# Autodesk Inventor assembly: Braço_robô_001
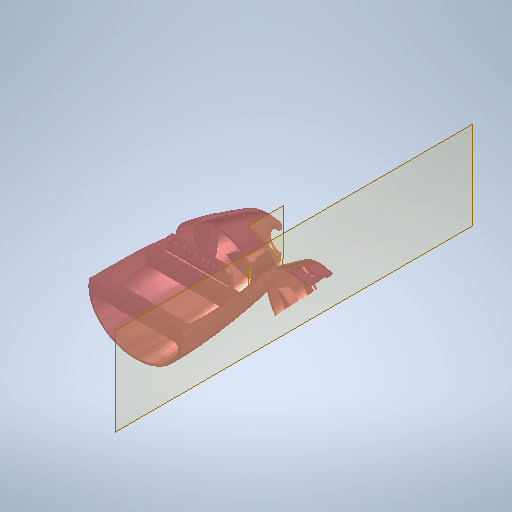
[picture p0: Inventor's stored thumbnail of the model, 512x512]
Saved by Autodesk Inventor 2025.2 (Build 292293000, 293)
## iProperties
Created: 2025-05-29
Part Number: Braço_robô_001
Document SubType Name: Assembly
Designer: Formação
Author: Formação
## Documents named in this file (8)
- C:\Users\Formação\Documents\Inventor\Mão_Robô_EMG\Mão Robótica 2.0\Braço_robô_001.iam
- C:\Users\Formação\Documents\Inventor\Mão_Robô_EMG\Mão Robótica 2.0\Braço\Mid Forearm Large.ipt
- C:\Users\Formação\Documents\Inventor\Mão_Robô_EMG\Mão Robótica 2.0\Braço\Mid Forearm Small.ipt
- C:\Users\Formação\Documents\Inventor\Mão_Robô_EMG\Mão Robótica 2.0\Braço\wrist clearance A.ipt
- C:\Users\Formação\Documents\Inventor\Mão_Robô_EMG\Mão Robótica 2.0\Braço\wrist clearance B.ipt
- C:\Users\Formação\Documents\Inventor\Mão_Robô_EMG\Mão Robótica 2.0\Braço\Wrist Forearm Section A.ipt
- C:\Users\Formação\Documents\Inventor\Mão_Robô_EMG\Mão Robótica 2.0\Braço\Wrist Forearm Section B.ipt
- C:\Users\Formação\Documents\Inventor\Mão_Robô_EMG\Mão Robótica 2.0\Palma\Palm _ Optimised Connector.ipt
## Components (7 placed, 7 different names)
1. Mid Forearm Large:1 — Coincidente:1, Coincidente:2, Coincidente:3, Coincidente:7, Coincidente:8, Coincidente:15, Coincidente:17, Coincidente:18, Coincidente:19, Coincidente:20
2. Mid Forearm Small:1 — Coincidente:15
3. wrist clearance A:1 — Coincidente:14, Coincidente:16
4. wrist clearance B:1 — Coincidente:10, Coincidente:11, Coincidente:14
5. Wrist Forearm Section A:1 — Coincidente:19, Coincidente:20, Coincidente:21, Ângulo:1
6. Wrist Forearm Section B:1 — Coincidente:7, Coincidente:8, Coincidente:10, Coincidente:11
7. Palm _ Optimised Connector:1 — Coincidente:16
## Relationships (17: Mate 16, Angle 1)
- Coincidente:1 [Mate]: Mid Forearm Large:1
- Coincidente:2 [Mate]: Mid Forearm Large:1
- Coincidente:3 [Mate]: Mid Forearm Large:1
- Coincidente:4 [Mate]
- Coincidente:7 [Mate]: Mid Forearm Large:1 ↔ Wrist Forearm Section B:1
- Coincidente:8 [Mate]: Mid Forearm Large:1 ↔ Wrist Forearm Section B:1
- Coincidente:10 [Mate]: wrist clearance B:1 ↔ Wrist Forearm Section B:1
- Coincidente:11 [Mate]: wrist clearance B:1 ↔ Wrist Forearm Section B:1
- Coincidente:14 [Mate]: wrist clearance A:1 ↔ wrist clearance B:1
- Coincidente:15 [Mate]: Mid Forearm Large:1 ↔ Mid Forearm Small:1
- Coincidente:16 [Mate] (51.985 mm): wrist clearance A:1 ↔ Palm _ Optimised Connector:1
- Coincidente:17 [Mate]: Mid Forearm Large:1
- Coincidente:18 [Mate]: Mid Forearm Large:1
- Coincidente:19 [Mate]: Mid Forearm Large:1 ↔ Wrist Forearm Section A:1
- Coincidente:20 [Mate]: Mid Forearm Large:1 ↔ Wrist Forearm Section A:1
- Coincidente:21 [Mate]: Wrist Forearm Section A:1
- Ângulo:1 [Angle] (0 deg): Wrist Forearm Section A:1
